# Autodesk Inventor assembly: Фиксатор правый
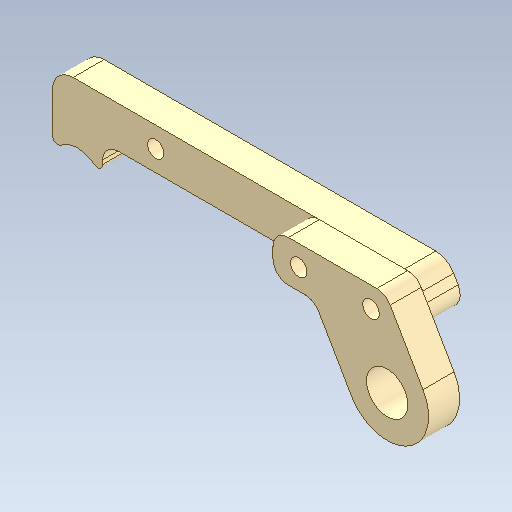
[picture p0: Inventor's stored thumbnail of the model, 512x512]
Saved by Autodesk Inventor 2021.1 (Build 251245010, 245A)
## iProperties
Created: 2026-04-16
Part Number: Фиксатор правый
Document SubType Name: Assembly
Designer: Андрей Тарасов
Author: Андрей Тарасов
## Documents named in this file (3)
- G:\04. Inventor\024. EDM 3.0\Система подачи и забора  проволоки\Фиксатор правый.iam
- G:\04. Inventor\024. EDM 3.0\Система подачи и забора  проволоки\Рычаг фиксатора 1.ipt
- G:\04. Inventor\024. EDM 3.0\Система подачи и забора  проволоки\Рычаг фиксатора 2.ipt
## Components (2 placed, 2 different names)
1. Рычаг фиксатора 1:1 — Совмещение:1, Совмещение:2, Совмещение:3
2. Рычаг фиксатора 2:1 — Совмещение:1, Совмещение:2, Совмещение:3
## Relationships (3: Mate 3)
- Совмещение:1 [Mate]: Рычаг фиксатора 1:1 ↔ Рычаг фиксатора 2:1
- Совмещение:2 [Mate]: Рычаг фиксатора 1:1 ↔ Рычаг фиксатора 2:1
- Совмещение:3 [Mate]: Рычаг фиксатора 1:1 ↔ Рычаг фиксатора 2:1
